# Autodesk Inventor assembly: Assy_power_module
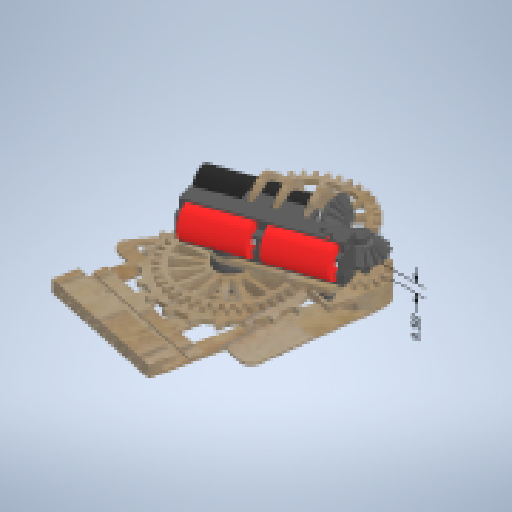
[picture p0: Inventor's stored thumbnail of the model, 512x512]
Saved by Autodesk Inventor 2026.1 (Build 301233020, 233B)
## iProperties
Created: 2025-09-27
Part Number: Assy_power_module
Document SubType Name: Assembly
Designer: hibik
Author: hibik
## Documents named in this file (17)
- C:\Users\hibik\Documents\Robomech\conveyer\power_module\Assy_power_module.iam
- C:\Users\hibik\Documents\Robomech\conveyer\power_module\gear_box.iam
- C:\Users\hibik\Documents\Robomech\conveyer\power_module\motor.ipt
- C:\Users\hibik\Documents\Robomech\conveyer\power_module\gear_plate_cover.ipt
- C:\Users\hibik\Documents\Robomech\conveyer\power_module\motor_setter_middle.ipt
- C:\Users\hibik\Documents\Robomech\conveyer\power_module\motor_setter_front.ipt
- C:\Users\hibik\Documents\Robomech\conveyer\power_module\motor_setter_fixer.ipt
- C:\Users\hibik\Documents\Robomech\conveyer\power_module\M3_15_crown_in.ipt
- C:\Users\hibik\Documents\Robomech\conveyer\power_module\battery_box.ipt
- C:\Users\hibik\Documents\Robomech\conveyer\power_module\battery.ipt
- C:\Users\hibik\Documents\Robomech\conveyer\power_module\nat_8.ipt
- C:\Users\hibik\Documents\Robomech\conveyer\power_module\nat_12.ipt
- C:\Users\hibik\Documents\Robomech\conveyer\power_module\spacer_wide.ipt
- C:\Users\hibik\Documents\Robomech\conveyer\power_module\spacer_2_hole.ipt
- C:\Users\hibik\Documents\Robomech\conveyer\power_module\nat_left.ipt
- C:\Users\hibik\Documents\Robomech\conveyer\power_module\nat_right.ipt
- C:\Users\hibik\Documents\Robomech\conveyer\power_module\nat_11.ipt
## Components (17 placed, 16 different names)
1. gear_box:1 [sub-assembly] — 挿入:1, 挿入:10, 挿入:15
2. motor:1 — 挿入:2, 挿入:3, 挿入:4
3. gear_plate_cover:1 — 挿入:1, メイト:4, メイト:5, メイト:6, メイト:7, 挿入:8, 挿入:9, 挿入:11, 挿入:12, 挿入:13
4. motor_setter_middle:1 — メイト:4, メイト:5, メイト:6, 挿入:2, 角度:1, メイト:8
5. motor_setter_front:1 — 挿入:3, 角度:1, 角度:2
6. motor_setter_fixer:1 — 挿入:4, 角度:2, 挿入:5, フラッシュ:1
7. M3_15_crown_in:1 — 挿入:5
8. battery_box:1 — メイト:7, メイト:8, フラッシュ:1, 挿入:6, 挿入:7
9. battery:1 — 挿入:6
10. battery:2 — 挿入:7
11. nat_8:1 — 挿入:8
12. nat_12:1 — 挿入:9
13. spacer_wide:1 — 挿入:10, 挿入:14
14. spacer_2_hole:1 — 挿入:11, 挿入:12
15. nat_left:1 — 挿入:13
16. nat_right:1 — 挿入:14
17. nat_11:1 — 挿入:15
## Relationships (23: Insert 15, Mate 5, Angle 2, Flush 1)
- 挿入:1 [Insert]: gear_box:1 ↔ gear_plate_cover:1
- メイト:4 [Mate]: gear_plate_cover:1 ↔ motor_setter_middle:1
- メイト:5 [Mate]: gear_plate_cover:1 ↔ motor_setter_middle:1
- メイト:6 [Mate]: gear_plate_cover:1 ↔ motor_setter_middle:1
- 挿入:2 [Insert] (-50 mm): motor:1 ↔ motor_setter_middle:1
- 挿入:3 [Insert]: motor:1 ↔ motor_setter_front:1
- 角度:1 [Angle] (0 deg): motor_setter_middle:1 ↔ motor_setter_front:1
- 挿入:4 [Insert]: motor:1 ↔ motor_setter_fixer:1
- 角度:2 [Angle] (0 deg): motor_setter_front:1 ↔ motor_setter_fixer:1
- 挿入:5 [Insert] (4.5 mm): motor_setter_fixer:1 ↔ M3_15_crown_in:1
- メイト:7 [Mate]: gear_plate_cover:1 ↔ battery_box:1
- メイト:8 [Mate]: motor_setter_middle:1 ↔ battery_box:1
- フラッシュ:1 [Flush] (-40 mm): motor_setter_fixer:1 ↔ battery_box:1
- 挿入:6 [Insert]: battery_box:1 ↔ battery:1
- 挿入:7 [Insert]: battery_box:1 ↔ battery:2
- 挿入:8 [Insert]: gear_plate_cover:1 ↔ nat_8:1
- 挿入:9 [Insert]: gear_plate_cover:1 ↔ nat_12:1
- 挿入:10 [Insert]: gear_box:1 ↔ spacer_wide:1
- 挿入:11 [Insert]: gear_plate_cover:1 ↔ spacer_2_hole:1
- 挿入:12 [Insert]: gear_plate_cover:1 ↔ spacer_2_hole:1
- 挿入:13 [Insert]: gear_plate_cover:1 ↔ nat_left:1
- 挿入:14 [Insert]: spacer_wide:1 ↔ nat_right:1
- 挿入:15 [Insert]: gear_box:1 ↔ nat_11:1
